# Autodesk Inventor assembly: Left arm
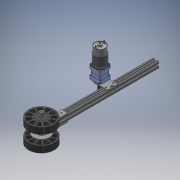
[picture p0: Inventor's stored thumbnail of the model, 180x180]
Saved by Autodesk Inventor 2018 (Build 220112000, 112)
## iProperties
Created: 2019-01-23
Part Number: Left arm
Document SubType Name: Assembly
Designer: s-2513225
Author: s-2513225
## Documents named in this file (8)
- E:\Robotics\ball intake 2018\Left arm.iam
- E:\Robotics\ball intake 2018\1010 16in.ipt
- E:\Robotics\ball intake 2018\VersaPlanetary_v1_Single_Stage_10_1_with_775_Series.ipt
- E:\Robotics\ball intake 2018\am-3480 4IN 500Hex Bore Compliant Wheel.ipt
- E:\Robotics\ball intake 2018\wheel tip.ipt
- E:\Robotics\ball intake 2018\0_500_ID_x_1_125_OD_x_0_313_WD_Flanged_Bearing_217-2731.ipt
- E:\Robotics\ball intake 2018\1_2_Hex_x_0_201_ID_ThunderHex_Stock_18_217-4002.ipt
- E:\Robotics\ball intake 2018\motor connector.ipt
## Components (10 placed, 7 different names)
1. 1010 16in:1 — Mate:1, Flush:1, Flush:2, Mate:2, Mate:10, Flush:6
2. VersaPlanetary_v1_Single_Stage_10_1_with_775_Series:1 — Mate:11, Mate:12
3. am-3480 4IN 500Hex Bore Compliant Wheel:1 — Mate:7, Mate:8
4. am-3480 4IN 500Hex Bore Compliant Wheel:2 — Mate:5, Mate:6
5. wheel tip:1 — Mate:1, Flush:1, Mate:3, Flush:3, Flush:5
6. wheel tip:2 — Flush:2, Mate:2, Mate:4, Flush:4, Flush:5
7. 0_500_ID_x_1_125_OD_x_0_313_WD_Flanged_Bearing_217-2731:1 — Mate:3, Flush:3, Mate:9
8. 0_500_ID_x_1_125_OD_x_0_313_WD_Flanged_Bearing_217-2731:2 — Mate:4, Flush:4
9. 1_2_Hex_x_0_201_ID_ThunderHex_Stock_18_217-4002:1 — Mate:5, Mate:6, Mate:7, Mate:8, Mate:9
10. motor connector:1 — Mate:10, Flush:6, Mate:11, Mate:12
## Relationships (18: Mate 12, Flush 6)
- Mate:1: 1010 16in:1 ↔ wheel tip:1
- Flush:1: 1010 16in:1 ↔ wheel tip:1
- Flush:2: 1010 16in:1 ↔ wheel tip:2
- Mate:2: 1010 16in:1 ↔ wheel tip:2
- Mate:3: wheel tip:1 ↔ 0_500_ID_x_1_125_OD_x_0_313_WD_Flanged_Bearing_217-2731:1
- Flush:3: wheel tip:1 ↔ 0_500_ID_x_1_125_OD_x_0_313_WD_Flanged_Bearing_217-2731:1
- Mate:4: wheel tip:2 ↔ 0_500_ID_x_1_125_OD_x_0_313_WD_Flanged_Bearing_217-2731:2
- Flush:4: wheel tip:2 ↔ 0_500_ID_x_1_125_OD_x_0_313_WD_Flanged_Bearing_217-2731:2
- Mate:5: am-3480 4IN 500Hex Bore Compliant Wheel:2 ↔ 1_2_Hex_x_0_201_ID_ThunderHex_Stock_18_217-4002:1
- Mate:6: am-3480 4IN 500Hex Bore Compliant Wheel:2 ↔ 1_2_Hex_x_0_201_ID_ThunderHex_Stock_18_217-4002:1
- Mate:7: am-3480 4IN 500Hex Bore Compliant Wheel:1 ↔ 1_2_Hex_x_0_201_ID_ThunderHex_Stock_18_217-4002:1
- Mate:8: am-3480 4IN 500Hex Bore Compliant Wheel:1 ↔ 1_2_Hex_x_0_201_ID_ThunderHex_Stock_18_217-4002:1
- Mate:9: 0_500_ID_x_1_125_OD_x_0_313_WD_Flanged_Bearing_217-2731:1 ↔ 1_2_Hex_x_0_201_ID_ThunderHex_Stock_18_217-4002:1
- Flush:5: wheel tip:1 ↔ wheel tip:2
- Mate:10: 1010 16in:1 ↔ motor connector:1
- Flush:6: 1010 16in:1 ↔ motor connector:1
- Mate:11: VersaPlanetary_v1_Single_Stage_10_1_with_775_Series:1 ↔ motor connector:1
- Mate:12: VersaPlanetary_v1_Single_Stage_10_1_with_775_Series:1 ↔ motor connector:1
